# Autodesk Inventor assembly: leg_motor_moudle_MIR
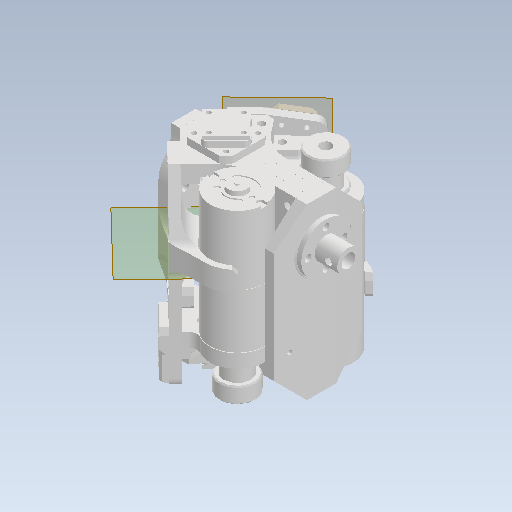
[picture p0: Inventor's stored thumbnail of the model, 512x512]
Saved by Autodesk Inventor 2020 (Build 240168000, 168)
## iProperties
Created: 2019-05-09
Part Number: leg_motor_moudle_MIR
Document SubType Name: Assembly
Designer: psrob
Author: psrob
## Documents named in this file (16)
- E:\projects-2\project dog gen2\hardware\leg_motor_moudle_MIR.iam
- E:\projects-2\project dog gen2\hardware\leg_basket_1_MIR.ipt
- E:\projects-2\project dog gen2\hardware\leg_basket_2_MIR.ipt
- E:\projects-2\project dog gen2\hardware\motor_holder_MIR.ipt
- E:\projects-2\project dog gen2\hardware\leg_basket_3_MIR.ipt
- E:\projects-2\project dog gen2\hardware\motor_2_MIR.ipt
- E:\projects-2\project dog gen2\hardware\pin_6_20_MIR.ipt
- E:\projects-2\project dog gen2\hardware\pin_6_60_MIR.ipt
- E:\projects-2\project dog gen2\hardware\2GT_wheel_MIR.ipt
- E:\projects-2\project dog gen2\hardware\bearing_6_13_5_MIR.ipt
- E:\projects-2\project dog gen2\hardware\flange_6mm_MIR.ipt
- E:\projects-2\project dog gen2\hardware\cross_axis_holder_1_MIR.ipt
- E:\projects-2\project dog gen2\hardware\2GT_wheel_5_MIR.ipt
- E:\projects-2\project dog gen2\hardware\encoder_ma1_MIR.ipt
- E:\projects-2\project dog gen2\hardware\encoder_ass_MIR1.iam
- E:\projects-2\project dog gen2\hardware\belt_holder_2_MIR.ipt
## Components (25 placed, 15 different names)
1. leg_basket_1_MIR:1 — Insert:6, Insert:5, Insert:8, Insert:7, Insert:2, Insert:1, Insert:4, Insert:3, Insert:29, Insert:28
2. leg_basket_2_MIR:1 — Insert:6, Insert:5, Insert:12, Insert:9, Insert:24, Insert:26, Insert:49, Insert:48
3. leg_basket_2_MIR:2 — Insert:8, Insert:7, Insert:11, Insert:10, Insert:25, Tangent:2, Mate:1, Insert:27, Insert:47, Insert:46
4. motor_holder_MIR:1 — Insert:2, Insert:1, Insert:20, Insert:19
5. motor_holder_MIR:2 — Insert:4, Insert:3, Insert:18, Insert:17
6. leg_basket_3_MIR:1 — Insert:12, Insert:11, Flush:1, Insert:55, Insert:54
7. leg_basket_3_MIR:2 — Insert:10, Insert:9, Insert:51, Insert:50
8. motor_2_MIR:1 — Insert:20, Insert:19, Insert:30
9. motor_2_MIR:2 — Insert:18, Insert:17, Insert:31
10. pin_6_20_MIR:1 — Insert:22, Insert:45
11. pin_6_60_MIR:1 — Insert:21, Insert:23, Tangent:1, Insert:44
12. 2GT_wheel_MIR:1 — Insert:21
13. bearing_6_13_5_MIR:1 — Insert:24, Insert:22
14. bearing_6_13_5_MIR:2 — Insert:25, Insert:23
15. flange_6mm_MIR:1 — Tangent:2, Tangent:1, Mate:1
16. cross_axis_holder_1_MIR:1 — Flush:1, Insert:27, Insert:26
17. flange_6mm_MIR:2 — Insert:29, Insert:28
18. 2GT_wheel_5_MIR:1 — Insert:31
19. 2GT_wheel_5_MIR:2 — Insert:30
20. encoder_ma1_MIR:1 — Insert:44
21. encoder_ma1_MIR:2 — Insert:45
22. encoder_ass_MIR1:1 [sub-assembly] — Insert:47, Insert:46
23. encoder_ass_MIR1:2 [sub-assembly] — Insert:49, Insert:48
24. belt_holder_2_MIR:1 — Insert:51, Insert:50
25. belt_holder_2_MIR:2 — Insert:55, Insert:54
## Relationships (41: Insert 37, Tangent 2, Mate 2)
- Insert:6: leg_basket_1_MIR:1 ↔ leg_basket_2_MIR:1
- Insert:5: leg_basket_1_MIR:1 ↔ leg_basket_2_MIR:1
- Insert:8: leg_basket_1_MIR:1 ↔ leg_basket_2_MIR:2
- Insert:7: leg_basket_1_MIR:1 ↔ leg_basket_2_MIR:2
- Insert:2: leg_basket_1_MIR:1 ↔ motor_holder_MIR:1
- Insert:1: leg_basket_1_MIR:1 ↔ motor_holder_MIR:1
- Insert:4: leg_basket_1_MIR:1 ↔ motor_holder_MIR:2
- Insert:3: leg_basket_1_MIR:1 ↔ motor_holder_MIR:2
- Insert:12: leg_basket_2_MIR:1 ↔ leg_basket_3_MIR:1
- Insert:11: leg_basket_2_MIR:2 ↔ leg_basket_3_MIR:1
- Insert:10: leg_basket_2_MIR:2 ↔ leg_basket_3_MIR:2
- Insert:9: leg_basket_2_MIR:1 ↔ leg_basket_3_MIR:2
- Insert:20: motor_holder_MIR:1 ↔ motor_2_MIR:1
- Insert:19: motor_holder_MIR:1 ↔ motor_2_MIR:1
- Insert:18: motor_holder_MIR:2 ↔ motor_2_MIR:2
- Insert:17: motor_holder_MIR:2 ↔ motor_2_MIR:2
- Insert:21 (-21 mm): pin_6_60_MIR:1 ↔ 2GT_wheel_MIR:1
- Insert:24: leg_basket_2_MIR:1 ↔ bearing_6_13_5_MIR:1
- Insert:22: pin_6_20_MIR:1 ↔ bearing_6_13_5_MIR:1
- Insert:25: leg_basket_2_MIR:2 ↔ bearing_6_13_5_MIR:2
- Insert:23: pin_6_60_MIR:1 ↔ bearing_6_13_5_MIR:2
- Tangent:2: leg_basket_2_MIR:2 ↔ flange_6mm_MIR:1
- Tangent:1: pin_6_60_MIR:1 ↔ flange_6mm_MIR:1
- Mate:1 (-5 mm): leg_basket_2_MIR:2 ↔ flange_6mm_MIR:1
- Flush:1 [Mate]: leg_basket_3_MIR:1 ↔ cross_axis_holder_1_MIR:1
- Insert:27: leg_basket_2_MIR:2 ↔ cross_axis_holder_1_MIR:1
- Insert:26: leg_basket_2_MIR:1 ↔ cross_axis_holder_1_MIR:1
- Insert:29: leg_basket_1_MIR:1 ↔ flange_6mm_MIR:2
- Insert:28: leg_basket_1_MIR:1 ↔ flange_6mm_MIR:2
- Insert:31 (-3 mm): motor_2_MIR:2 ↔ 2GT_wheel_5_MIR:1
- Insert:30 (-3 mm): motor_2_MIR:1 ↔ 2GT_wheel_5_MIR:2
- Insert:44: pin_6_60_MIR:1 ↔ encoder_ma1_MIR:1
- Insert:45: pin_6_20_MIR:1 ↔ encoder_ma1_MIR:2
- Insert:47: leg_basket_2_MIR:2 ↔ encoder_ass_MIR1:1
- Insert:46: leg_basket_2_MIR:2 ↔ encoder_ass_MIR1:1
- Insert:49: leg_basket_2_MIR:1 ↔ encoder_ass_MIR1:2
- Insert:48: leg_basket_2_MIR:1 ↔ encoder_ass_MIR1:2
- Insert:51: leg_basket_3_MIR:2 ↔ belt_holder_2_MIR:1
- Insert:50: leg_basket_3_MIR:2 ↔ belt_holder_2_MIR:1
- Insert:55: leg_basket_3_MIR:1 ↔ belt_holder_2_MIR:2
- Insert:54: leg_basket_3_MIR:1 ↔ belt_holder_2_MIR:2
